# Autodesk Inventor assembly: 细轴四方中间洞
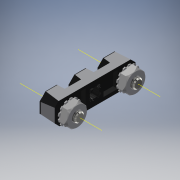
[picture p0: Inventor's stored thumbnail of the model, 180x180]
Saved by Autodesk Inventor 2019.4 (Build 234330000, 330)
## iProperties
Created: 2019-05-20
Part Number: 细轴四方中间洞
Material: 常规
Document SubType Name: Assembly
Designer: aresp
Author: aresp
## Documents named in this file (4)
- D:\2019-2020TowerTakeOverCad\ncrCadLib\细轴四方中间洞.iam
- D:\2019-2020TowerTakeOverCad\ncrCadLib\轴相关\细轴四方轴承\四方轴套.ipt
- D:\2019-2020TowerTakeOverCad\ncrCadLib\轴相关\细轴四方轴承.ipt
- D:\2019-2020TowerTakeOverCad\ncrCadLib\细轴四方轴套用的螺丝螺帽套.iam
## Components (3 placed, 2 different names)
1. 四方轴套:1 — 配合:4
2. 细轴四方轴套用的螺丝螺帽套:1 [sub-assembly] — 表面齐平:1
3. 细轴四方轴套用的螺丝螺帽套:2 [sub-assembly] — 表面齐平:1, 配合:4
## Relationships (4: Mate 3, Flush 1)
- [Mate]: 四方轴套:1 ↔ 细轴四方轴套用的螺丝螺帽套:1
- [Mate]: 四方轴套:1 ↔ 细轴四方轴套用的螺丝螺帽套:1
- 表面齐平:1 [Flush]: 细轴四方轴套用的螺丝螺帽套:1 ↔ 细轴四方轴套用的螺丝螺帽套:2
- 配合:4 [Mate]: 四方轴套:1 ↔ 细轴四方轴套用的螺丝螺帽套:2
